# Autodesk Inventor assembly: pitch-frame
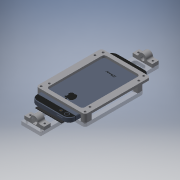
[picture p0: Inventor's stored thumbnail of the model, 180x180]
Saved by Autodesk Inventor 2016 (Build 200138000, 138)
## iProperties
Created: 2015-12-01
Part Number: pitch-frame
Document SubType Name: Assembly
Designer: jufranz
Author: jufranz
## Documents named in this file (6)
- C:\Users\jfranz\Documents\GitHub\perspection\hardware\cad\pitch-frame.iam
- C:\Users\jfranz\Documents\GitHub\perspection\hardware\cad\phone_plate.ipt
- C:\Users\jfranz\Documents\GitHub\perspection\hardware\cad\motor_bracket.ipt
- C:\Users\jfranz\Documents\GitHub\perspection\hardware\cad\apple-iphone-5-7.snapshot.1\iPhone 5 (Black).iam
- C:\Users\jfranz\Documents\GitHub\perspection\hardware\cad\phone_cushion.ipt
- C:\Users\jfranz\Documents\GitHub\perspection\hardware\cad\phone_clamp_v2.ipt
## Components (6 placed, 5 different names)
1. phone_plate:1 — Insert:1, Insert:2, Insert:3, Insert:4, Mate:1, Insert:5, Insert:6
2. motor_bracket:1 — Insert:1, Insert:2
3. motor_bracket:2 — Insert:3, Insert:4
4. iPhone 5 (Black):1 [sub-assembly] — Mate:2
5. phone_cushion:1 — Mate:1, Mate:2
6. phone_clamp_v2:1 — Insert:5, Insert:6
## Relationships (8: Insert 6, Mate 2)
- Insert:1: phone_plate:1 ↔ motor_bracket:1
- Insert:2: phone_plate:1 ↔ motor_bracket:1
- Insert:3: phone_plate:1 ↔ motor_bracket:2
- Insert:4: phone_plate:1 ↔ motor_bracket:2
- Mate:1: phone_plate:1 ↔ phone_cushion:1
- Mate:2: iPhone 5 (Black):1 ↔ phone_cushion:1
- Insert:5: phone_plate:1 ↔ phone_clamp_v2:1
- Insert:6: phone_plate:1 ↔ phone_clamp_v2:1
